# Autodesk Inventor assembly: MicroGimbal Assembly
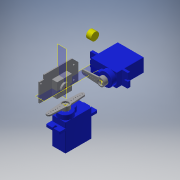
[picture p0: Inventor's stored thumbnail of the model, 180x180]
Saved by Autodesk Inventor 2016 (Build 200138000, 138)
## iProperties
Created: 2016-02-12
Part Number: MicroGimbal Assembly
Document SubType Name: Assembly
Designer: RoksBot
Author: RoksBot
## Documents named in this file (6)
- C:\Users\RoksBot\Documents\Inventor\Camera Mount\MicroGimbal Assembly.iam
- C:\Users\RoksBot\Documents\Inventor\Camera Mount\MicroServo Horn.ipt
- C:\Users\RoksBot\Documents\Inventor\Camera Mount\MicroServo.ipt
- C:\Users\RoksBot\Documents\Inventor\Camera Mount\Camera.ipt
- C:\Users\RoksBot\Documents\Inventor\Camera Mount\2 Way MicroServo Attachment.ipt
- C:\Users\RoksBot\Documents\Inventor\Camera Mount\1 Way MicroServo Attachment.ipt
## Components (7 placed, 5 different names)
1. MicroServo Horn:1 — Insert:1, Pan RL, Flush:1, Mate:1, Insert:3, Mate:3
2. MicroServo:1 — Insert:1, Pan RL
3. MicroServo Horn:2 — Insert:2, Pan UD, Mate:2, Insert:4, Flush:2
4. MicroServo:2 — Insert:2, Pan UD, Mate:4
5. Camera:1 — Flush:1, Mate:1, Mate:2, Mate:5
6. 2 Way MicroServo Attachment:1 — Insert:3, Mate:3, Mate:4
7. 1 Way MicroServo Attachment:1 — Insert:4, Flush:2, Mate:5
## Relationships (13: Mate 5, Insert 4, Angle 2, Flush 2)
- Insert:1: MicroServo Horn:1 ↔ MicroServo:1
- Insert:2: MicroServo Horn:2 ↔ MicroServo:2
- Pan RL [Angle] (0 deg): MicroServo Horn:1 ↔ MicroServo:1
- Pan UD [Angle] (0 deg): MicroServo Horn:2 ↔ MicroServo:2
- Flush:1: MicroServo Horn:1 ↔ Camera:1
- Mate:1: MicroServo Horn:1 ↔ Camera:1
- Mate:2: MicroServo Horn:2 ↔ Camera:1
- Insert:3: MicroServo Horn:1 ↔ 2 Way MicroServo Attachment:1
- Mate:3: MicroServo Horn:1 ↔ 2 Way MicroServo Attachment:1
- Insert:4: MicroServo Horn:2 ↔ 1 Way MicroServo Attachment:1
- Flush:2: MicroServo Horn:2 ↔ 1 Way MicroServo Attachment:1
- Mate:4 (5.715 mm): MicroServo:2 ↔ 2 Way MicroServo Attachment:1
- Mate:5 (2.54 mm): Camera:1 ↔ 1 Way MicroServo Attachment:1
